# Autodesk Inventor assembly: CH3-chassisFull
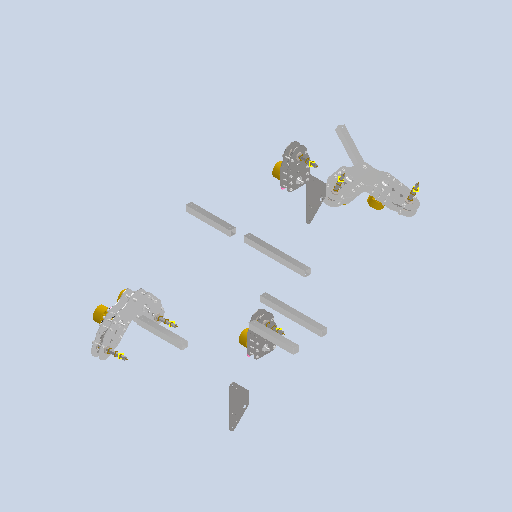
[picture p0: Inventor's stored thumbnail of the model, 512x512]
Saved by Autodesk Inventor 2025.1 (Build 291241020, 241B)
## iProperties
Created: 2025-01-30
Part Number: CH3-chassisFull
Document SubType Name: Assembly
Designer: t205b
Author: t205b
## Documents named in this file (8)
- C:\Users\t205b\OneDrive\Documents\Github\BehrendURCMechanical\CAD\Chassis V3\CH3-chassisFull.iam
- C:\Users\t205b\OneDrive\Documents\Github\BehrendURCMechanical\CAD\Chassis V3\aluminumextrusiontool\aluminumextrusiontool-17-10.6in.ipt
- C:\Users\t205b\OneDrive\Documents\Github\BehrendURCMechanical\CAD\Chassis V3\aluminumextrusiontool.ipt
- C:\Users\t205b\OneDrive\Documents\Github\BehrendURCMechanical\CAD\Chassis V3\aluminumextrusiontool\aluminumextrusiontool-17-7.9.ipt
- C:\Users\t205b\OneDrive\Documents\Github\BehrendURCMechanical\CAD\Chassis V3\CH3-L3DoubleGearbox.iam
- C:\Users\t205b\OneDrive\Documents\Github\BehrendURCMechanical\CAD\Chassis V3\CH3-L1SingleGearbox.iam
- C:\Users\t205b\OneDrive\Documents\Github\BehrendURCMechanical\CAD\Chassis V3\HipPivotPlate.ipt
- C:\Users\t205b\OneDrive\Documents\Github\BehrendURCMechanical\CAD\Chassis V3\CH3-PivotBoltNutWasher.iam
## Components (14 placed, 6 different names)
1. aluminumextrusiontool-17-10.6in:2
2. aluminumextrusiontool-17-7.9:3
3. aluminumextrusiontool-17-7.9:4
4. aluminumextrusiontool-17-7.9:5
5. aluminumextrusiontool-17-7.9:6 — Mate:3
6. aluminumextrusiontool-17-10.6in:7
7. CH3-L3DoubleGearbox:1 [sub-assembly] — Mate:1, Mate:2
8. CH3-L3DoubleGearbox:2 [sub-assembly] — Mate:4, Mate:5
9. CH3-L1SingleGearbox:1 [sub-assembly]
10. CH3-L1SingleGearbox:2 [sub-assembly]
11. HipPivotPlate:1
12. HipPivotPlate:2
13. CH3-PivotBoltNutWasher:1 [sub-assembly] — Mate:1, Mate:2
14. CH3-PivotBoltNutWasher:2 [sub-assembly] — Mate:3, Mate:4, Mate:5
## Relationships (5: Mate 5)
- Mate:1: CH3-L3DoubleGearbox:1 ↔ CH3-PivotBoltNutWasher:1
- Mate:2: CH3-L3DoubleGearbox:1 ↔ CH3-PivotBoltNutWasher:1
- Mate:3: aluminumextrusiontool-17-7.9:6 ↔ CH3-PivotBoltNutWasher:2
- Mate:4: CH3-L3DoubleGearbox:2 ↔ CH3-PivotBoltNutWasher:2
- Mate:5: CH3-L3DoubleGearbox:2 ↔ CH3-PivotBoltNutWasher:2
